# Autodesk Inventor assembly: Deploy_assembly
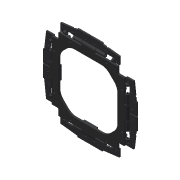
[picture p0: Inventor's stored thumbnail of the model, 180x180]
Saved by Autodesk Inventor 2019.4 (Build 234330000, 330)
## iProperties
Created: 2020-01-06
Part Number: Deploy_assembly
Material: Genérico
Document SubType Name: Assembly
Designer: Elias
Author: Elias
## Documents named in this file (3)
- C:\Users\Elias\Google Drive (els.obrq@gmail.com)\Archivos CAD\Satellites\Payloads SUCHAI 2&3\Articulacion\Fabricacion Windform\Deploy_assembly.iam
- C:\Users\Elias\Google Drive (els.obrq@gmail.com)\Archivos CAD\Satellites\Payloads SUCHAI 2&3\Articulacion\Fabricacion Windform\SoportePlaca_SPEL_Rev.3.ipt
- C:\Users\Elias\Google Drive (els.obrq@gmail.com)\Archivos CAD\Satellites\Payloads SUCHAI 2&3\Articulacion\Fabricacion Windform\SoporteUNION_SPEL_Rev.1.ipt
## Components (5 placed, 2 different names)
1. SoportePlaca_SPEL_Rev.3:1 — Coincidencia:7, Coincidencia:8, Ángulo:4
2. SoporteUNION_SPEL_Rev.1:1 — Coincidencia:1, Coincidencia:2, Ángulo:1, Coincidencia:3, Coincidencia:4, Ángulo:2, Coincidencia:5, Coincidencia:6, Ángulo:3, Coincidencia:7, Coincidencia:8, Ángulo:4
3. SoportePlaca_SPEL_Rev.3:2 — Coincidencia:1, Coincidencia:2, Ángulo:1
4. SoportePlaca_SPEL_Rev.3:3 — Coincidencia:3, Coincidencia:4, Ángulo:2
5. SoportePlaca_SPEL_Rev.3:4 — Coincidencia:5, Coincidencia:6, Ángulo:3
## Relationships (12: Mate 8, Angle 4)
- Coincidencia:1 [Mate]: SoporteUNION_SPEL_Rev.1:1 ↔ SoportePlaca_SPEL_Rev.3:2
- Coincidencia:2 [Mate] (0.5 mm): SoporteUNION_SPEL_Rev.1:1 ↔ SoportePlaca_SPEL_Rev.3:2
- Ángulo:1 [Angle] (0 deg): SoporteUNION_SPEL_Rev.1:1 ↔ SoportePlaca_SPEL_Rev.3:2
- Coincidencia:3 [Mate]: SoporteUNION_SPEL_Rev.1:1 ↔ SoportePlaca_SPEL_Rev.3:3
- Coincidencia:4 [Mate] (0.5 mm): SoporteUNION_SPEL_Rev.1:1 ↔ SoportePlaca_SPEL_Rev.3:3
- Ángulo:2 [Angle] (0 deg): SoporteUNION_SPEL_Rev.1:1 ↔ SoportePlaca_SPEL_Rev.3:3
- Coincidencia:5 [Mate]: SoporteUNION_SPEL_Rev.1:1 ↔ SoportePlaca_SPEL_Rev.3:4
- Coincidencia:6 [Mate] (0.5 mm): SoporteUNION_SPEL_Rev.1:1 ↔ SoportePlaca_SPEL_Rev.3:4
- Ángulo:3 [Angle] (0 deg): SoporteUNION_SPEL_Rev.1:1 ↔ SoportePlaca_SPEL_Rev.3:4
- Coincidencia:7 [Mate]: SoportePlaca_SPEL_Rev.3:1 ↔ SoporteUNION_SPEL_Rev.1:1
- Coincidencia:8 [Mate] (0.5 mm): SoportePlaca_SPEL_Rev.3:1 ↔ SoporteUNION_SPEL_Rev.1:1
- Ángulo:4 [Angle] (0 deg): SoportePlaca_SPEL_Rev.3:1 ↔ SoporteUNION_SPEL_Rev.1:1
